# Autodesk Inventor assembly: tank_assembly
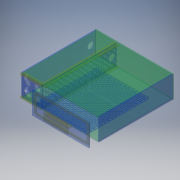
[picture p0: Inventor's stored thumbnail of the model, 180x180]
Saved by Autodesk Inventor 2018.1 (Build 221171000, 171)
## iProperties
Created: 2017-07-30
Part Number: tank_assembly
Document SubType Name: Assembly
Designer: Tom
Mass: 2878.67 g
Surface Area: 12320.6 cm^2
Volume: 2056.19 cm^3
Density: 1.4 g/cm^3
Author: Tom
## Documents named in this file (9)
- \\Mac\Dropbox\2015-2016\Bachelorproef\Inventor\Etstank_v2\tank_assembly.iam
- \\Mac\Dropbox\2015-2016\Bachelorproef\Inventor\Etstank_v2\tank_bottom.ipt
- \\Mac\Dropbox\2015-2016\Bachelorproef\Inventor\Etstank_v2\tank_side.ipt
- \\Mac\Dropbox\2015-2016\Bachelorproef\Inventor\Etstank_v2\tank_front.ipt
- \\Mac\Dropbox\2015-2016\Bachelorproef\Inventor\Etstank_v2\tank_back.ipt
- \\Mac\Dropbox\2015-2016\Bachelorproef\Inventor\Etstank_v2\tank_separator_assembly.iam
- \\Mac\Dropbox\2015-2016\Bachelorproef\Inventor\Etstank_v2\tank_sensorssupport_assembly.iam
- \\Mac\Dropbox\2015-2016\Bachelorproef\Inventor\Etstank_v2\tank_lid_assembly.iam
- \\Mac\Dropbox\2015-2016\Bachelorproef\Inventor\Etstank_v2\par.xls
## Components (8 placed, 7 different names)
1. tank_bottom:1 — Flush:2, Mate:1, Flush:3, Flush:4, Mate:3, Flush:5, Mate:4, Mate:6
2. tank_side:1 — Flush:2, Mate:1, Flush:3, Flush:7, Flush:10, Flush:12, Lift
3. tank_side:2 — Flush:4, Mate:3, Flush:5, Mate:5, Flush:6, Mate:7
4. tank_front:1 — Mate:4, Mate:5, Flush:6, Flush:11
5. tank_back:1 — Mate:6, Mate:7, Flush:7, Mate:9, Mate:10
6. tank_separator_assembly:1 [sub-assembly] — Mate:8, Flush:8, Flush:9
7. tank_sensorssupport_assembly:1 [sub-assembly] — Mate:8, Flush:8, Flush:9, Mate:9, Mate:10, Flush:10
8. tank_lid_assembly:1 [sub-assembly] — Flush:11, Flush:12, Lift
## Relationships (21: Flush 11, Mate 10)
- Flush:2 (5 mm): tank_bottom:1 ↔ tank_side:1
- Mate:1: tank_bottom:1 ↔ tank_side:1
- Flush:3: tank_bottom:1 ↔ tank_side:1
- Flush:4 (5 mm): tank_bottom:1 ↔ tank_side:2
- Mate:3: tank_bottom:1 ↔ tank_side:2
- Flush:5: tank_bottom:1 ↔ tank_side:2
- Mate:4: tank_bottom:1 ↔ tank_front:1
- Mate:5: tank_side:2 ↔ tank_front:1
- Flush:6: tank_side:2 ↔ tank_front:1
- Mate:6: tank_bottom:1 ↔ tank_back:1
- Mate:7: tank_side:2 ↔ tank_back:1
- Flush:7: tank_side:1 ↔ tank_back:1
- Mate:8: tank_separator_assembly:1 ↔ tank_sensorssupport_assembly:1
- Flush:8: tank_separator_assembly:1 ↔ tank_sensorssupport_assembly:1
- Flush:9: tank_separator_assembly:1 ↔ tank_sensorssupport_assembly:1
- Mate:9: tank_back:1 ↔ tank_sensorssupport_assembly:1
- Mate:10: tank_back:1 ↔ tank_sensorssupport_assembly:1
- Flush:10: tank_side:1 ↔ tank_sensorssupport_assembly:1
- Flush:11: tank_front:1 ↔ tank_lid_assembly:1
- Flush:12: tank_side:1 ↔ tank_lid_assembly:1
- Lift [Mate]: tank_side:1 ↔ tank_lid_assembly:1
## Named parameters: maxh = 400 mm, maxw = 350 mm, lcsd = 19.05 mm, lcdd = 100 mm, lcwd1 = 25 mm, lcwd2 = 34 mm, lcw = 20 mm, lch1 = 39 mm, lch2 = 40 mm, lcl = 150 mm, lcwd3 = 43 mm, dia1 = 6 mm, td = 18 mm, bhh = 6 mm, bhd = 10 mm, sw = 25 mm, sh = 31 mm, spacert = 2 mm, nutdist = 40 mm, platft = 20 mm, supt = 20 mm, pvct = 5 mm, tankw = 100 mm, tankh = 370 mm, tankl = 379 mm, dia2 = 20 mm, tankv = 1e+07 mm, actual_tankv = 1.4023e+07 mm, dia3 = 8 mm, dia4 = 11 mm, play = 9 mm, holeh = 26 mm, surroundh = 60 mm, slack = 0.5 mm, surroundt = 5 mm, play2 = 3 mm, maxl = 400 mm, diaoverflow = 25 mm, diacucl = 32 mm, extra_height = 100 mm, diaph = 32 mm, diaair = 32 mm, diawater = 25 mm, mindist = 80 mm, distfromedge = 10 mm, diasurroundhole = 42 mm, diagrate = 12 mm, brachetw = 10 mm, sensorsupportl = 100 mm, gratespacing = 12.02082 mm, sidedist = 13.9375 mm, bottomdist = 9.6355 mm, diafloat = 50 mm, diahcl = 32 mm, bracketw = 10 mm, bracketwtop = 6 mm, bracketwbottom = 6 mm, handlesupporth = 20 mm, handlew = 50 mm, handlel = 120 mm, nett = 1 mm, nethole = 16 mm, netside = 3.5 mm, nettop = 7 mm, netholespacing = 2 mm, nutholdert = 10 mm, diaetape = 32 mm
